# Autodesk Inventor assembly: 1717_SR+16A_PAIR
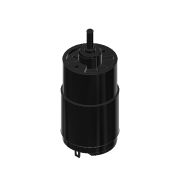
[picture p0: Inventor's stored thumbnail of the model, 180x180]
Saved by Autodesk Inventor 2019.4 (Build 234330000, 330)
## iProperties
Created: 2019-10-19
Part Number: 1717_SR+16A_PAIR
Material: 一般
Document SubType Name: Assembly
Designer: y6tada
Author: y6tada
## Documents named in this file (3)
- C:\GrabCAD\Yunit 8\Libs\1717_SR+16A_PAIR.iam
- C:\GrabCAD\Yunit 8\Libs\1717_SR_3D-CAD\1717T_SR.ipt
- C:\GrabCAD\Yunit 8\Libs\16A_3D-CAD\16A_3STAGE.ipt
## Components (2 placed, 2 different names)
1. 1717T_SR:1 — メイト:1, メイト:2
2. 16A_3STAGE:1 — メイト:1, メイト:2, メイト:3
## Relationships (3: Mate 3)
- メイト:1 [Mate]: 1717T_SR:1 ↔ 16A_3STAGE:1
- メイト:2 [Mate]: 1717T_SR:1 ↔ 16A_3STAGE:1
- メイト:3 [Mate]: 16A_3STAGE:1
